# Autodesk Inventor assembly: outer
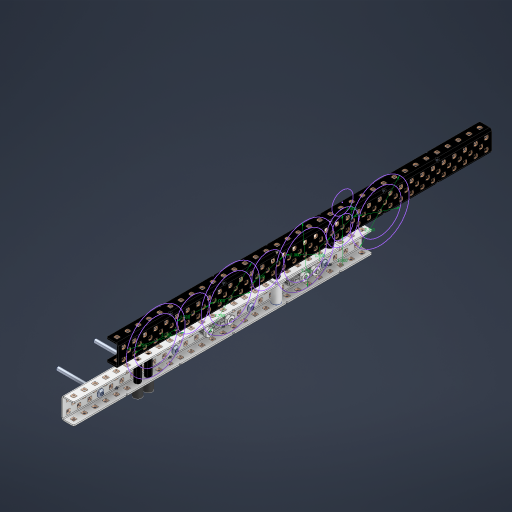
[picture p0: Inventor's stored thumbnail of the model, 512x512]
Saved by Autodesk Inventor 2024 (Build 280153000, 153)
## iProperties
Created: 2023-10-18
Part Number: outer
Document SubType Name: Assembly
Designer: avere
Author: avere
## Documents named in this file (13)
- C:\Users\avere\Documents\rbp_cad\goated_v0.1\chassis\drivebay\outer.iam
- C:\Users\avere\Documents\rbp_cad\VEX-CAD-Inventor-1.41\Structure\C Channel\Aluminum 1x2x1\Alu C 1x2x1x35.ipt
- C:\Users\avere\Documents\rbp_cad\VEX-CAD-Inventor-1.41\Structure\C Channel\Aluminum 1x2x1\Alu C 1x2x1x28.ipt
- C:\Users\avere\Documents\rbp_cad\VEX-CAD-Inventor-1.41\Structure\C Channel\Aluminum 1x2x1\Alu C 1x2x1x6.ipt
- C:\Users\avere\Documents\rbp_cad\VEX-CAD-Inventor-1.41\lightweight_offset_bearing.iam
- C:\Users\avere\Documents\rbp_cad\hardware\.375 OD Aluminum Spacer 0.875.ipt
- C:\Users\avere\Documents\rbp_cad\VEX-CAD-Inventor-1.41\Structure\Standoff\Standoff .875.ipt
- C:\Users\avere\Documents\rbp_cad\VEX-CAD-Inventor-1.41\Structure\Standoff.ipt
- C:\Users\avere\Documents\rbp_cad\VEX-CAD-Inventor-1.41\lightweight_bearing.iam
- C:\Users\avere\Documents\rbp_cad\VEX-CAD-Inventor-1.41\Motion\Spacers\Spacer Nylon .375 OD\NSpacer .375 OD x .500.ipt
- C:\Users\avere\Documents\rbp_cad\VEX-CAD-Inventor-1.41\Motion\Spacers\Spacer Nylon .375 OD.ipt
- C:\Users\avere\Documents\rbp_cad\VEX-CAD-Inventor-1.41\Structure\Hardware\Screw Shoulder Robosource\SScrew Shoulder Smooth 2.000 x .04.ipt
- C:\Users\avere\Documents\rbp_cad\VEX-CAD-Inventor-1.41\Structure\Hardware\Screw Shoulder Robosource.ipt
## Components (18 placed, 9 different names)
1. Alu C 1x2x1x35:1
2. Alu C 1x2x1x28:1 — Insert:1, Mate:1, Insert:3, Insert:7, Mate:3, Insert:8, Mate:4, Insert:9, Insert:10, Insert:11, Insert:12, Insert:13, Insert:14, Insert:15, Insert:16, Insert:17
3. Alu C 1x2x1x6:1 — Insert:1, Mate:1, Insert:2, Mate:2, Insert:5, Insert:6
4. lightweight_offset_bearing:1 [sub-assembly] — Insert:2, Mate:2
5. .375 OD Aluminum Spacer 0.875:1 — Insert:3
6. Standoff .875:1 — Insert:5
7. Standoff .875:2 — Insert:6
8. lightweight_offset_bearing:2 [sub-assembly] — Insert:7, Mate:3
9. lightweight_bearing:1 [sub-assembly] — Insert:8, Mate:4
10. NSpacer .375 OD x .500:1 — Insert:9
11. NSpacer .375 OD x .500:2 — Insert:10
12. Standoff .875:3 — Insert:11
13. Standoff .875:4 — Insert:12
14. SScrew Shoulder Smooth 2.000 x .04:1 — Insert:13
15. SScrew Shoulder Smooth 2.000 x .04:2 — Insert:14
16. SScrew Shoulder Smooth 2.000 x .04:3 — Insert:15
17. SScrew Shoulder Smooth 2.000 x .04:4 — Insert:16
18. SScrew Shoulder Smooth 2.000 x .04:5 — Insert:17
## Relationships (20: Insert 16, Mate 4)
- Insert:1: Alu C 1x2x1x28:1 ↔ Alu C 1x2x1x6:1
- Mate:1: Alu C 1x2x1x28:1 ↔ Alu C 1x2x1x6:1
- Insert:2: Alu C 1x2x1x6:1 ↔ lightweight_offset_bearing:1
- Mate:2: Alu C 1x2x1x6:1 ↔ lightweight_offset_bearing:1
- Insert:3: Alu C 1x2x1x28:1 ↔ .375 OD Aluminum Spacer 0.875:1
- Insert:5: Alu C 1x2x1x6:1 ↔ Standoff .875:1
- Insert:6: Alu C 1x2x1x6:1 ↔ Standoff .875:2
- Insert:7: Alu C 1x2x1x28:1 ↔ lightweight_offset_bearing:2
- Mate:3: Alu C 1x2x1x28:1 ↔ lightweight_offset_bearing:2
- Insert:8: Alu C 1x2x1x28:1 ↔ lightweight_bearing:1
- Mate:4: Alu C 1x2x1x28:1 ↔ lightweight_bearing:1
- Insert:9: Alu C 1x2x1x28:1 ↔ NSpacer .375 OD x .500:1
- Insert:10: Alu C 1x2x1x28:1 ↔ NSpacer .375 OD x .500:2
- Insert:11: Alu C 1x2x1x28:1 ↔ Standoff .875:3
- Insert:12: Alu C 1x2x1x28:1 ↔ Standoff .875:4
- Insert:13: Alu C 1x2x1x28:1 ↔ SScrew Shoulder Smooth 2.000 x .04:1
- Insert:14: Alu C 1x2x1x28:1 ↔ SScrew Shoulder Smooth 2.000 x .04:2
- Insert:15: Alu C 1x2x1x28:1 ↔ SScrew Shoulder Smooth 2.000 x .04:3
- Insert:16: Alu C 1x2x1x28:1 ↔ SScrew Shoulder Smooth 2.000 x .04:4
- Insert:17: Alu C 1x2x1x28:1 ↔ SScrew Shoulder Smooth 2.000 x .04:5
